# Autodesk Inventor assembly: intakeStealthSub
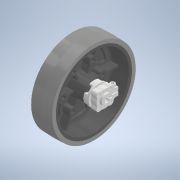
[picture p0: Inventor's stored thumbnail of the model, 180x180]
Saved by Autodesk Inventor 2020 (Build 240168000, 168)
## iProperties
Created: 2019-10-18
Part Number: intakeStealthSub
Document SubType Name: Assembly
Designer: tdmp4
Author: tdmp4
## Documents named in this file (4)
- C:\Users\tdmp4\OneDrive\Documents\GitHub\CAD-2020\Intake\intakeStealthSub.iam
- C:\Users\tdmp4\OneDrive\Documents\GitHub\CAD-2020\AndyMark\am-2648 4inWheel 8mm Hub REV2.ipt
- C:\Users\tdmp4\OneDrive\Documents\GitHub\CAD-2020\ServoCity\545456.ipt
- C:\Users\tdmp4\OneDrive\Documents\GitHub\CAD-2020\ServoCity\545619 assembly.ipt
## Components (3 placed, 3 different names)
1. am-2648 4inWheel 8mm Hub REV2:1 — Mate:1, Mate:5
2. 545456:1 — Mate:1, Mate:5, Mate:6, Mate:7, Mate:8
3. 545619 assembly:1 — Mate:6, Mate:7, Mate:8
## Relationships (5: Mate 5)
- Mate:1: am-2648 4inWheel 8mm Hub REV2:1 ↔ 545456:1
- Mate:5: am-2648 4inWheel 8mm Hub REV2:1 ↔ 545456:1
- Mate:6: 545456:1 ↔ 545619 assembly:1
- Mate:7: 545456:1 ↔ 545619 assembly:1
- Mate:8: 545456:1 ↔ 545619 assembly:1
